# Autodesk Inventor assembly: Servo_ver2
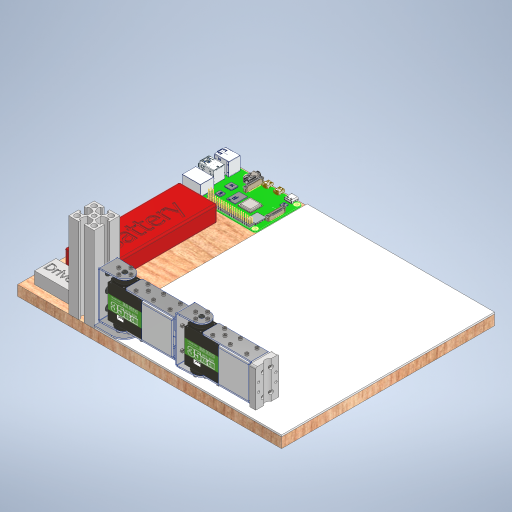
[picture p0: Inventor's stored thumbnail of the model, 512x512]
Saved by Autodesk Inventor 2023 (Build 270158000, 158)
## iProperties
Created: 2022-10-22
Part Number: Servo_ver2
Document SubType Name: Assembly
Designer: 박동준
Author: 박동준
## Documents named in this file (23)
- C:\Users\chanh\OneDrive - 연세대학교 (Yonsei University)\로봇\Humanoid\Roboin Humanoid Project\Inventor\2-Axis Manipulator\Designs\Assembly\Servo_ver2.iam
- C:\Users\chanh\OneDrive - 연세대학교 (Yonsei University)\로봇\Humanoid\Roboin Humanoid Project\Inventor\2-Axis Manipulator\Designs\Part\base_plate.ipt
- C:\Users\chanh\OneDrive - 연세대학교 (Yonsei University)\로봇\Humanoid\Roboin Humanoid Project\Inventor\2-Axis Manipulator\Designs\Part\servo_bracket_bottom.ipt
- C:\Users\chanh\OneDrive - 연세대학교 (Yonsei University)\로봇\Humanoid\Roboin Humanoid Project\Inventor\2-Axis Manipulator\Designs\Part\servo_bracket_top.ipt
- C:\Users\chanh\OneDrive - 연세대학교 (Yonsei University)\로봇\Humanoid\Roboin Humanoid Project\Inventor\2-Axis Manipulator\Designs\Part\servo-horn_bottom.ipt
- C:\Users\chanh\OneDrive - 연세대학교 (Yonsei University)\로봇\Humanoid\Roboin Humanoid Project\Inventor\2-Axis Manipulator\Designs\Part\servo-horn_top.ipt
- C:\Users\chanh\OneDrive - 연세대학교 (Yonsei University)\로봇\Humanoid\Roboin Humanoid Project\Inventor\2-Axis Manipulator\Designs\Part\servo.ipt
- C:\Users\chanh\OneDrive - 연세대학교 (Yonsei University)\로봇\Humanoid\Roboin Humanoid Project\Inventor\2-Axis Manipulator\Designs\Part\ㄷ_frame_1.ipt
- C:\Users\chanh\OneDrive - 연세대학교 (Yonsei University)\로봇\Humanoid\Roboin Humanoid Project\Inventor\2-Axis Manipulator\Designs\Part\3030 Aluminium Profile.ipt
- C:\Users\chanh\OneDrive - 연세대학교 (Yonsei University)\로봇\Humanoid\Roboin Humanoid Project\Inventor\2-Axis Manipulator\Designs\Part\ㄷ_frame_2.ipt
- C:\Users\chanh\OneDrive - 연세대학교 (Yonsei University)\로봇\Humanoid\Roboin Humanoid Project\Inventor\2-Axis Manipulator\Designs\Part\Frame_Bottom_Plate.ipt
- C:\Users\chanh\OneDrive - 연세대학교 (Yonsei University)\로봇\Humanoid\Roboin Humanoid Project\Inventor\2-Axis Manipulator\Designs\Part\Raspberry Pi, Motor Driver, Battery\Raspberry Pi 4 Model B.iam
- C:\Users\chanh\OneDrive - 연세대학교 (Yonsei University)\로봇\Humanoid\Roboin Humanoid Project\Inventor\2-Axis Manipulator\Designs\Part\Raspberry Pi, Motor Driver, Battery\Battery Pack.ipt
- C:\Users\chanh\OneDrive - 연세대학교 (Yonsei University)\로봇\Humanoid\Roboin Humanoid Project\Inventor\2-Axis Manipulator\Designs\Part\Raspberry Pi, Motor Driver, Battery\Motor Driver.ipt
- C:\Users\chanh\OneDrive - 연세대학교 (Yonsei University)\로봇\Humanoid\Roboin Humanoid Project\Inventor\2-Axis Manipulator\Designs\Part\M4x10 볼트.ipt
- C:\Users\chanh\OneDrive - 연세대학교 (Yonsei University)\로봇\Humanoid\Roboin Humanoid Project\Inventor\2-Axis Manipulator\Designs\Part\M6x30 볼트.ipt
- C:\Users\chanh\OneDrive - 연세대학교 (Yonsei University)\로봇\Humanoid\Roboin Humanoid Project\Inventor\2-Axis Manipulator\Designs\Part\acryl plate.ipt
- C:\Users\chanh\OneDrive - 연세대학교 (Yonsei University)\로봇\Humanoid\Roboin Humanoid Project\Inventor\2-Axis Manipulator\Designs\Part\ㄷ_frame_3.ipt
- C:\Users\chanh\OneDrive - 연세대학교 (Yonsei University)\로봇\Humanoid\Roboin Humanoid Project\Inventor\2-Axis Manipulator\Designs\Part\M2x4 볼트.ipt
- C:\Users\chanh\OneDrive - 연세대학교 (Yonsei University)\로봇\Humanoid\Roboin Humanoid Project\Inventor\2-Axis Manipulator\Designs\Part\M3x6 볼트.ipt
- C:\Users\chanh\OneDrive - 연세대학교 (Yonsei University)\로봇\Humanoid\Roboin Humanoid Project\Inventor\2-Axis Manipulator\Designs\Part\M3x5 볼트.ipt
- C:\Users\chanh\OneDrive - 연세대학교 (Yonsei University)\로봇\Humanoid\Roboin Humanoid Project\Inventor\2-Axis Manipulator\Designs\Part\end_arm_수정.ipt
- C:\Users\chanh\OneDrive - 연세대학교 (Yonsei University)\로봇\Humanoid\Roboin Humanoid Project\Inventor\2-Axis Manipulator\Designs\Part\M2x6 볼트.ipt
## Components (86 placed, 22 different names)
1. M2x4 볼트:41 — Rigid:78
2. M2x4 볼트:40 — Rigid:79
3. M2x4 볼트:39 — Rigid:80
4. M2x4 볼트:38 — Rigid:81
5. M2x4 볼트:37 — Rigid:77
6. M2x4 볼트:36 — Rigid:76
7. M2x4 볼트:35 — Rigid:75
8. M2x4 볼트:34 — Rigid:74
9. M2x4 볼트:33 — Rigid:82
10. M2x4 볼트:32 — Rigid:83
11. M2x4 볼트:31 — Rigid:71
12. M2x4 볼트:30 — Rigid:70
13. M2x4 볼트:29 — Rigid:85
14. M2x4 볼트:28 — Rigid:84
15. M2x4 볼트:27 — Rigid:73
16. M2x4 볼트:26 — Rigid:72
17. M2x4 볼트:42 — Rigid:49
18. M2x4 볼트:25 — Rigid:50
19. M2x4 볼트:24 — Rigid:48
20. M2x4 볼트:23 — Rigid:47
21. M2x4 볼트:22 — Rigid:46
22. M2x4 볼트:21 — Rigid:45
23. M2x4 볼트:20 — Rigid:44
24. M2x4 볼트:19 — Rigid:103
25. M2x4 볼트:18 — Rigid:100
26. M2x4 볼트:17 — Rigid:102
27. M2x4 볼트:16 — Rigid:101
28. M2x4 볼트:15 — Rigid:95
29. M2x4 볼트:14 — Rigid:97
30. M2x4 볼트:13 — Rigid:98
31. M2x4 볼트:12 — Rigid:96
32. M2x4 볼트:11 — Rigid:93
33. M2x4 볼트:10 — Rigid:94
34. M2x4 볼트:9 — Rigid:92
35. M2x4 볼트:8 — Rigid:91
36. M2x4 볼트:7 — Rigid:26
37. M2x4 볼트:6 — Rigid:25
38. M2x4 볼트:5 — Rigid:24
39. M2x4 볼트:4 — Rigid:23
40. M2x4 볼트:3 — Rigid:22
41. M2x4 볼트:2 — Rigid:21
42. M2x4 볼트:1 — Rigid:20
43. M2x4 볼트:43 — Rigid:61
44. M2x4 볼트:44 — Rigid:63
45. M2x4 볼트:45 — Rigid:60
46. M2x4 볼트:46 — Rigid:62
47. M2x4 볼트:47 — Rigid:16, Mate:9
48. M2x4 볼트:48 — Rigid:18
49. M2x4 볼트:49 — Rigid:17
50. M2x4 볼트:50 — Rigid:65
51. M2x6 볼트:1 — Rigid:106
52. M2x6 볼트:2 — Rigid:107
53. M2x6 볼트:3 — Rigid:108
54. M2x6 볼트:4 — Rigid:109
55. M3x5 볼트:1 — Rigid:88
56. M3x5 볼트:2 — Rigid:89
57. M3x6 볼트:1 — Rigid:86
58. M3x6 볼트:2 — Rigid:87
59. M4x10 볼트:1 — Rigid:58
60. M4x10 볼트:2 — Rigid:55
61. M4x10 볼트:3 — Rigid:56
62. M6x30 볼트:1 — Rigid:57
63. ㄷ_frame_3:1 — Rigid:66
64. ㄷ_frame_3:2 — Rigid:67
65. ㄷ_frame_3:3 — Rigid:69
66. ㄷ_frame_3:4 — Rigid:68
67. Frame_Bottom_Plate:1 — Mate:7, Flush:5, Mate:9, Mate:14
68. servo_bracket_bottom:3 — Rigid:43, Rigid:47, Rigid:48, Rigid:49, Rigid:50, Rigid:78, Rigid:79, Rigid:80, Rigid:81
69. servo_bracket_top:3 — Rigid:42, Rigid:44, Rigid:45, Rigid:46, Rigid:68, Rigid:69, Rigid:74, Rigid:75, Rigid:76, Rigid:77, Rigid:105
70. ㄷ_frame_2:1 — Rigid:90, Rigid:91, Rigid:92, Rigid:93, Rigid:94, Rigid:95, Rigid:96, Rigid:97, Rigid:98, Rigid:99, Rigid:100, Rigid:101, Rigid:102, Rigid:103, Rigid:104
71. servo_bracket_top:2 — 강체:3, Rigid:20, Rigid:21, Rigid:22, Rigid:66, Rigid:67, Rigid:70, Rigid:71, Rigid:72, Rigid:73, Rigid:90
72. servo_bracket_bottom:2 — 강체:4, Rigid:23, Rigid:24, Rigid:25, Rigid:26, Rigid:82, Rigid:83, Rigid:84, Rigid:85
73. ㄷ_frame_1:1 — 플러쉬:4, 메이트:4, Rigid:16, Rigid:17, Rigid:18, Rigid:55, Rigid:56, Rigid:58, Rigid:59, Rigid:60, Rigid:61, Rigid:62, Rigid:63, Rigid:64, Rigid:65
74. servo-horn_bottom:3 — Rigid:99
75. servo-horn_top:3 — Rotational:2, Rigid:87, Rigid:104
76. servo:2 — Rotational:2, Rigid:42, Rigid:43, Rigid:89
77. servo:1 — Rotational:1, 강체:3, 강체:4, Rigid:88
78. servo-horn_bottom:2 — Rigid:64
79. servo-horn_top:2 — Rotational:1, Rigid:59, Rigid:86
80. end_arm_수정:1 — Rigid:105, Rigid:106, Rigid:107, Rigid:108, Rigid:109
81. acryl plate:1 — Mate:13, Flush:15, Flush:16, Mate:14
82. Motor Driver:1 — Mate:12, Flush:9, Flush:10
83. Battery Pack:1 — Mate:11, Flush:11, Flush:12
84. base_plate:1 — Flush:6, Flush:7, Flush:8, Rigid:52, Mate:10, Mate:11, Mate:12, Flush:9, Flush:10, Flush:11, Flush:12, Flush:13, Flush:14, Rigid:57, Mate:13, Flush:15, Flush:16
85. Raspberry Pi 4 Model B:1 [sub-assembly] — Mate:10, Flush:13, Flush:14
86. 3030 Aluminium Profile:1 — 플러쉬:4, 메이트:4, Mate:7, Flush:5, Rigid:52
## Relationships (100: WeldJoint 77, Flush 13, Mate 8, RevoluteJoint 2)
- Rotational:1 [RevoluteJoint] (0.9 mm): servo:1 ↔ servo-horn_top:2
- 강체:3 [WeldJoint]: servo_bracket_top:2 ↔ servo:1
- 강체:4 [WeldJoint]: servo_bracket_bottom:2 ↔ servo:1
- 플러쉬:4 [Flush]: ㄷ_frame_1:1 ↔ 3030 Aluminium Profile:1
- 메이트:4 [Mate]: ㄷ_frame_1:1 ↔ 3030 Aluminium Profile:1
- Rigid:16 [WeldJoint]: M2x4 볼트:47 ↔ ㄷ_frame_1:1
- Rigid:17 [WeldJoint]: M2x4 볼트:49 ↔ ㄷ_frame_1:1
- Rigid:18 [WeldJoint]: M2x4 볼트:48 ↔ ㄷ_frame_1:1
- Rigid:20 [WeldJoint]: M2x4 볼트:1 ↔ servo_bracket_top:2
- Rigid:21 [WeldJoint]: M2x4 볼트:2 ↔ servo_bracket_top:2
- Rigid:22 [WeldJoint]: M2x4 볼트:3 ↔ servo_bracket_top:2
- Rigid:23 [WeldJoint]: M2x4 볼트:4 ↔ servo_bracket_bottom:2
- Rigid:24 [WeldJoint]: M2x4 볼트:5 ↔ servo_bracket_bottom:2
- Rigid:25 [WeldJoint]: M2x4 볼트:6 ↔ servo_bracket_bottom:2
- Rigid:26 [WeldJoint]: M2x4 볼트:7 ↔ servo_bracket_bottom:2
- Rotational:2 [RevoluteJoint] (0.9 mm): servo-horn_top:3 ↔ servo:2
- Rigid:42 [WeldJoint]: servo_bracket_top:3 ↔ servo:2
- Rigid:43 [WeldJoint]: servo_bracket_bottom:3 ↔ servo:2
- Rigid:44 [WeldJoint]: M2x4 볼트:20 ↔ servo_bracket_top:3
- Rigid:45 [WeldJoint]: M2x4 볼트:21 ↔ servo_bracket_top:3
- Rigid:46 [WeldJoint]: M2x4 볼트:22 ↔ servo_bracket_top:3
- Rigid:47 [WeldJoint]: M2x4 볼트:23 ↔ servo_bracket_bottom:3
- Rigid:48 [WeldJoint]: M2x4 볼트:24 ↔ servo_bracket_bottom:3
- Rigid:49 [WeldJoint]: M2x4 볼트:42 ↔ servo_bracket_bottom:3
- Rigid:50 [WeldJoint]: M2x4 볼트:25 ↔ servo_bracket_bottom:3
- Mate:7: Frame_Bottom_Plate:1 ↔ 3030 Aluminium Profile:1
- Flush:5: Frame_Bottom_Plate:1 ↔ 3030 Aluminium Profile:1
- Flush:6: base_plate:1
- Flush:7: base_plate:1
- Flush:8: base_plate:1
- Rigid:52 [WeldJoint]: base_plate:1 ↔ 3030 Aluminium Profile:1
- Mate:9: M2x4 볼트:47 ↔ Frame_Bottom_Plate:1
- Mate:10 (1.4 mm): base_plate:1 ↔ Raspberry Pi 4 Model B:1
- Mate:11: Battery Pack:1 ↔ base_plate:1
- Mate:12: Motor Driver:1 ↔ base_plate:1
- Flush:9 (10 mm): Motor Driver:1 ↔ base_plate:1
- Flush:10 (-10 mm): Motor Driver:1 ↔ base_plate:1
- Flush:11 (-10 mm): Battery Pack:1 ↔ base_plate:1
- Flush:12 (70 mm): Battery Pack:1 ↔ base_plate:1
- Flush:13 (190 mm): base_plate:1 ↔ Raspberry Pi 4 Model B:1
- Flush:14 (4 mm): base_plate:1 ↔ Raspberry Pi 4 Model B:1
- Rigid:55 [WeldJoint]: M4x10 볼트:2 ↔ ㄷ_frame_1:1
- Rigid:56 [WeldJoint]: M4x10 볼트:3 ↔ ㄷ_frame_1:1
- Rigid:57 [WeldJoint]: M6x30 볼트:1 ↔ base_plate:1
- Rigid:58 [WeldJoint]: M4x10 볼트:1 ↔ ㄷ_frame_1:1
- Rigid:59 [WeldJoint]: ㄷ_frame_1:1 ↔ servo-horn_top:2
- Rigid:60 [WeldJoint]: M2x4 볼트:45 ↔ ㄷ_frame_1:1
- Rigid:61 [WeldJoint]: M2x4 볼트:43 ↔ ㄷ_frame_1:1
- Rigid:62 [WeldJoint]: M2x4 볼트:46 ↔ ㄷ_frame_1:1
- Rigid:63 [WeldJoint]: M2x4 볼트:44 ↔ ㄷ_frame_1:1
- Rigid:64 [WeldJoint]: ㄷ_frame_1:1 ↔ servo-horn_bottom:2
- Rigid:65 [WeldJoint]: M2x4 볼트:50 ↔ ㄷ_frame_1:1
- Mate:13: acryl plate:1 ↔ base_plate:1
- Flush:15: acryl plate:1 ↔ base_plate:1
- Flush:16: acryl plate:1 ↔ base_plate:1
- Mate:14: Frame_Bottom_Plate:1 ↔ acryl plate:1
- Rigid:66 [WeldJoint]: ㄷ_frame_3:1 ↔ servo_bracket_top:2
- Rigid:67 [WeldJoint]: ㄷ_frame_3:2 ↔ servo_bracket_top:2
- Rigid:68 [WeldJoint]: ㄷ_frame_3:4 ↔ servo_bracket_top:3
- Rigid:69 [WeldJoint]: ㄷ_frame_3:3 ↔ servo_bracket_top:3
- Rigid:70 [WeldJoint]: M2x4 볼트:30 ↔ servo_bracket_top:2
- Rigid:71 [WeldJoint]: M2x4 볼트:31 ↔ servo_bracket_top:2
- Rigid:72 [WeldJoint]: M2x4 볼트:26 ↔ servo_bracket_top:2
- Rigid:73 [WeldJoint]: M2x4 볼트:27 ↔ servo_bracket_top:2
- Rigid:74 [WeldJoint]: M2x4 볼트:34 ↔ servo_bracket_top:3
- Rigid:75 [WeldJoint]: M2x4 볼트:35 ↔ servo_bracket_top:3
- Rigid:76 [WeldJoint]: M2x4 볼트:36 ↔ servo_bracket_top:3
- Rigid:77 [WeldJoint]: M2x4 볼트:37 ↔ servo_bracket_top:3
- Rigid:78 [WeldJoint]: M2x4 볼트:41 ↔ servo_bracket_bottom:3
- Rigid:79 [WeldJoint]: M2x4 볼트:40 ↔ servo_bracket_bottom:3
- Rigid:80 [WeldJoint]: M2x4 볼트:39 ↔ servo_bracket_bottom:3
- Rigid:81 [WeldJoint]: M2x4 볼트:38 ↔ servo_bracket_bottom:3
- Rigid:82 [WeldJoint]: M2x4 볼트:33 ↔ servo_bracket_bottom:2
- Rigid:83 [WeldJoint]: M2x4 볼트:32 ↔ servo_bracket_bottom:2
- Rigid:84 [WeldJoint]: M2x4 볼트:28 ↔ servo_bracket_bottom:2
- Rigid:85 [WeldJoint]: M2x4 볼트:29 ↔ servo_bracket_bottom:2
- Rigid:86 [WeldJoint]: M3x6 볼트:1 ↔ servo-horn_top:2
- Rigid:87 [WeldJoint]: M3x6 볼트:2 ↔ servo-horn_top:3
- Rigid:88 [WeldJoint]: M3x5 볼트:1 ↔ servo:1
- Rigid:89 [WeldJoint]: M3x5 볼트:2 ↔ servo:2
- Rigid:90 [WeldJoint]: ㄷ_frame_2:1 ↔ servo_bracket_top:2
- Rigid:91 [WeldJoint]: M2x4 볼트:8 ↔ ㄷ_frame_2:1
- Rigid:92 [WeldJoint]: M2x4 볼트:9 ↔ ㄷ_frame_2:1
- Rigid:93 [WeldJoint]: M2x4 볼트:11 ↔ ㄷ_frame_2:1
- Rigid:94 [WeldJoint]: M2x4 볼트:10 ↔ ㄷ_frame_2:1
- Rigid:95 [WeldJoint]: M2x4 볼트:15 ↔ ㄷ_frame_2:1
- Rigid:96 [WeldJoint]: M2x4 볼트:12 ↔ ㄷ_frame_2:1
- Rigid:97 [WeldJoint]: M2x4 볼트:14 ↔ ㄷ_frame_2:1
- Rigid:98 [WeldJoint]: M2x4 볼트:13 ↔ ㄷ_frame_2:1
- Rigid:99 [WeldJoint]: ㄷ_frame_2:1 ↔ servo-horn_bottom:3
- Rigid:100 [WeldJoint]: M2x4 볼트:18 ↔ ㄷ_frame_2:1
- Rigid:101 [WeldJoint]: M2x4 볼트:16 ↔ ㄷ_frame_2:1
- Rigid:102 [WeldJoint]: M2x4 볼트:17 ↔ ㄷ_frame_2:1
- Rigid:103 [WeldJoint]: M2x4 볼트:19 ↔ ㄷ_frame_2:1
- Rigid:104 [WeldJoint]: ㄷ_frame_2:1 ↔ servo-horn_top:3
- Rigid:105 [WeldJoint]: servo_bracket_top:3 ↔ end_arm_수정:1
- Rigid:106 [WeldJoint]: M2x6 볼트:1 ↔ end_arm_수정:1
- Rigid:107 [WeldJoint]: M2x6 볼트:2 ↔ end_arm_수정:1
- Rigid:108 [WeldJoint]: M2x6 볼트:3 ↔ end_arm_수정:1
- Rigid:109 [WeldJoint]: M2x6 볼트:4 ↔ end_arm_수정:1
